# Autodesk Inventor assembly: Gornja_konstrukcija_s_držačima_assembly
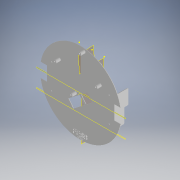
[picture p0: Inventor's stored thumbnail of the model, 180x180]
Saved by Autodesk Inventor 2020 (Build 240168000, 168)
## iProperties
Created: 2020-10-14
Part Number: Gornja_konstrukcija_s_držačima_assembly
Document SubType Name: Assembly
Designer: Sičaja
Author: Sičaja
## Documents named in this file (3)
- C:\Users\Sicaja\Documents\Projects\3D Drawings\Inventor_draws\Robocup\Inverntor_parts_for_print\Gornja_konstrukcija_s_držačima_assembly.iam
- C:\Users\Sicaja\Documents\Projects\3D Drawings\Inventor_draws\Robocup\Inverntor_parts_for_print\GornjaKonstrukcija_lidari_kamere_v.2.0.ipt
- C:\Users\Sicaja\Documents\Projects\3D Drawings\Inventor_draws\Robocup\Inverntor_parts_for_print\5DržačaLidara.ipt
## Components (3 placed, 2 different names)
1. GornjaKonstrukcija_lidari_kamere_v.2.0:1 — Mate:1, Mate:2, Flush:2
2. 5DržačaLidara:1 — Mate:1, Mate:2, Flush:1
3. 5DržačaLidara:2
## Component patterns: (2 elements, first: 5DržačaLidara:1)
## Relationships (4: Mate 2, Flush 2)
- Mate:1: GornjaKonstrukcija_lidari_kamere_v.2.0:1 ↔ 5DržačaLidara:1
- Mate:2: GornjaKonstrukcija_lidari_kamere_v.2.0:1 ↔ 5DržačaLidara:1
- Flush:1 (6.8 mm): 5DržačaLidara:1
- Flush:2: GornjaKonstrukcija_lidari_kamere_v.2.0:1
